# Autodesk Inventor assembly: full
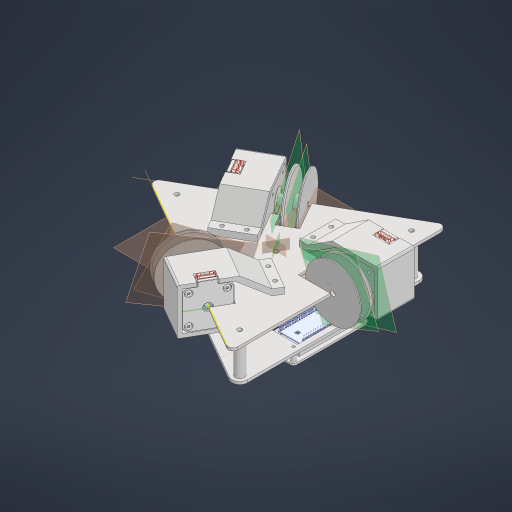
[picture p0: Inventor's stored thumbnail of the model, 512x512]
Saved by Autodesk Inventor 2024 (Build 280153000, 153)
## iProperties
Created: 2026-03-23
Part Number: full
Document SubType Name: Assembly
Designer: schar
Author: schar
## Documents named in this file (10)
- C:\Users\schar\Desktop\FloatingFace\models\full.iam
- C:\Users\schar\Desktop\FloatingFace\models\baseplate.ipt
- C:\Users\schar\Desktop\FloatingFace\models\spool.ipt
- C:\Users\schar\Desktop\FloatingFace\models\17HS4401S_Stepper_Motor\17HS4401S_Stepper_Motor.iam
- C:\Users\schar\Desktop\FloatingFace\models\esp32-s3-wroom-1-1.snapshot.2\ESP32-S3-WROOM-1\ESP32-S3-WROOM-1.iam
- C:\Users\schar\Desktop\FloatingFace\models\nema_brackets_and_lineguides.ipt
- C:\Users\schar\3D Objects\spacer_etage.ipt
- C:\Users\schar\3D Objects\second_etage.ipt
- C:\Users\schar\3D Objects\esp_spacer_fixed.ipt
- C:\Users\schar\Desktop\FloatingFace\models\esp_plate.ipt
## Components (20 placed, 9 different names)
1. baseplate:1 — Mate:1, Mate:2, Mate:3, Mate:11, Mate:12, Flush:1, Mate:13, Mate:14, Mate:15, Flush:2, Flush:3, Flush:11, Flush:13, Mate:18, Mate:19, Mate:20, Mate:21, Flush:15, Mate:22, Mate:23
2. spool:1 — Mate:1, Mate:2, Mate:4, Mate:5
3. 17HS4401S_Stepper_Motor:1 [sub-assembly] — Mate:3, Mate:4, Mate:5
4. ESP32-S3-WROOM-1:1 [sub-assembly] — Mate:32, Flush:18, Flush:19
5. spool:2
6. 17HS4401S_Stepper_Motor:4 [sub-assembly] — Mate:14, Mate:15, Flush:2, Mate:16, Mate:17
7. spool:3 — Mate:11, Flush:4
8. 17HS4401S_Stepper_Motor:5 [sub-assembly] — Mate:12, Flush:1, Mate:13
9. nema_brackets_and_lineguides:1 — Flush:3, Flush:4, Flush:10
10. nema_brackets_and_lineguides:2 — Mate:16, Flush:11, Mate:17, Flush:12
11. spacer_etage:1 — Flush:13
12. spacer_etage:2 — Mate:18, Mate:19, Flush:14, Mate:31
13. spacer_etage:3 — Mate:20, Mate:21
14. second_etage:1 — Flush:14, Flush:16, Mate:25, Mate:26, Mate:27, Mate:28, Mate:29, Mate:30, Mate:31
15. nema_brackets_and_lineguides:3 — Flush:15, Mate:22, Mate:23
16. esp_spacer_fixed:1 — Flush:16, Flush:17
17. esp_spacer_fixed:2 — Mate:25, Mate:30
18. esp_spacer_fixed:3 — Mate:26, Mate:29
19. esp_spacer_fixed:4 — Mate:27, Mate:28
20. esp_plate:1 — Flush:17, Mate:32, Flush:18, Flush:19
## Relationships (44: Mate 30, Flush 14)
- Mate:1: baseplate:1 ↔ spool:1
- Mate:2: baseplate:1 ↔ spool:1
- Mate:3: baseplate:1 ↔ 17HS4401S_Stepper_Motor:1
- Mate:4: spool:1 ↔ 17HS4401S_Stepper_Motor:1
- Mate:5: spool:1 ↔ 17HS4401S_Stepper_Motor:1
- [Mate]: spool:2 ↔ 17HS4401S_Stepper_Motor:4
- [Mate]: spool:2 ↔ 17HS4401S_Stepper_Motor:4
- [Mate]: spool:3 ↔ 17HS4401S_Stepper_Motor:5
- [Mate]: spool:3 ↔ 17HS4401S_Stepper_Motor:5
- Mate:11: baseplate:1 ↔ spool:3
- Mate:12: baseplate:1 ↔ 17HS4401S_Stepper_Motor:5
- Flush:1: baseplate:1 ↔ 17HS4401S_Stepper_Motor:5
- Mate:13: baseplate:1 ↔ 17HS4401S_Stepper_Motor:5
- Mate:14: baseplate:1 ↔ 17HS4401S_Stepper_Motor:4
- Mate:15: baseplate:1 ↔ 17HS4401S_Stepper_Motor:4
- Flush:2: baseplate:1 ↔ 17HS4401S_Stepper_Motor:4
- Flush:3: baseplate:1 ↔ nema_brackets_and_lineguides:1
- Flush:4 (2 mm): spool:3 ↔ nema_brackets_and_lineguides:1
- Flush:10: nema_brackets_and_lineguides:1
- Mate:16: 17HS4401S_Stepper_Motor:4 ↔ nema_brackets_and_lineguides:2
- Flush:11: baseplate:1 ↔ nema_brackets_and_lineguides:2
- Mate:17: 17HS4401S_Stepper_Motor:4 ↔ nema_brackets_and_lineguides:2
- Flush:12: nema_brackets_and_lineguides:2
- Flush:13: baseplate:1 ↔ spacer_etage:1
- Mate:18: baseplate:1 ↔ spacer_etage:2
- Mate:19: baseplate:1 ↔ spacer_etage:2
- Mate:20: baseplate:1 ↔ spacer_etage:3
- Mate:21: baseplate:1 ↔ spacer_etage:3
- Flush:14: spacer_etage:2 ↔ second_etage:1
- Flush:15: baseplate:1 ↔ nema_brackets_and_lineguides:3
- Mate:22: baseplate:1 ↔ nema_brackets_and_lineguides:3
- Mate:23: baseplate:1 ↔ nema_brackets_and_lineguides:3
- Flush:16: second_etage:1 ↔ esp_spacer_fixed:1
- Mate:25: second_etage:1 ↔ esp_spacer_fixed:2
- Mate:26: second_etage:1 ↔ esp_spacer_fixed:3
- Mate:27: second_etage:1 ↔ esp_spacer_fixed:4
- Mate:28: second_etage:1 ↔ esp_spacer_fixed:4
- Mate:29: second_etage:1 ↔ esp_spacer_fixed:3
- Mate:30: second_etage:1 ↔ esp_spacer_fixed:2
- Mate:31: spacer_etage:2 ↔ second_etage:1
- Flush:17: esp_spacer_fixed:1 ↔ esp_plate:1
- Mate:32: ESP32-S3-WROOM-1:1 ↔ esp_plate:1
- Flush:18: ESP32-S3-WROOM-1:1 ↔ esp_plate:1
- Flush:19: ESP32-S3-WROOM-1:1 ↔ esp_plate:1
## Named parameters: d8_d5 = 0 mm, d9_d6 = 0 mm, d10_d5 = 0 mm, d11_d6 = 0 mm
